# Autodesk Inventor assembly: Base Cover Assembly
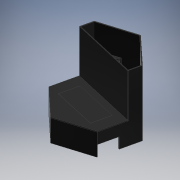
[picture p0: Inventor's stored thumbnail of the model, 180x180]
Saved by Autodesk Inventor 2017 (Build 210142000, 142)
## iProperties
Created: 2018-10-18
Part Number: Base Cover Assembly
Document SubType Name: Assembly
Designer: Dell
Author: Dell
## Documents named in this file (12)
- C:\Users\Dell\Documents\GitHub\tr2\Base\Base Cover Assembly.iam
- C:\Users\Dell\Documents\GitHub\tr2\Base\BA03.ipt
- C:\Users\Dell\Documents\GitHub\tr2\Base\BA04.ipt
- C:\Users\Dell\Documents\GitHub\tr2\Base\BA05.ipt
- C:\Users\Dell\Documents\GitHub\tr2\Base\BA10.ipt
- C:\Users\Dell\Documents\GitHub\tr2\Base\BA14.ipt
- C:\Users\Dell\Documents\GitHub\tr2\Base\BA19.ipt
- C:\Users\Dell\Documents\GitHub\tr2\Base\BA25.ipt
- C:\Users\Dell\Documents\GitHub\tr2\Base\BA26.ipt
- C:\Users\Dell\Documents\GitHub\tr2\Base\BA27.ipt
- C:\Users\Dell\slaterobots.com\Slate Robotics OneDrive - Documents\Autodesk Inventor\tr2-rs1\Base\HDMI Port.ipt
- C:\Users\Dell\slaterobots.com\Slate Robotics OneDrive - Documents\Autodesk Inventor\tr2-rs1\Base\Power Switch\Power Switch.iam
## Components (12 placed, 11 different names)
1. BA04:1 — Mate:7, Mate:8, Flush:1, Flush:4, Mate:12, Flush:8, Mate:22
2. BA05:1 — Mate:5, Mate:6, Flush:3, Mate:13, Mate:20, Flush:9, Mate:21
3. BA03:5 — Flush:2, Flush:3, Mate:18, Mate:21
4. BA10:1 — Mate:3, Mate:4, Mate:6, Mate:8, Flush:7, Mate:14, Mate:15, Mate:16, Mate:17, Mate:20
5. BA14:1 — Flush:1, Flush:2, Mate:18, Mate:22, Mate:23, Mate:24, Mate:25
6. BA19:2 — Flush:4, Mate:12, Mate:13, Flush:8, Flush:9
7. BA25:1 — Mate:1, Mate:4, Mate:7, Mate:17
8. BA25:2 — Mate:1, Mate:3, Mate:5, Mate:16
9. BA26:1 — Flush:7, Mate:14, Mate:15
10. BA27:1 — Mate:23, Mate:24, Mate:25, Mate:26, Mate:27, Angle:1, Mate:28, Mate:29, Flush:10
11. HDMI Port:1 — Mate:28, Mate:29, Flush:10
12. Power Switch:1 [sub-assembly] — Mate:26, Mate:27, Angle:1
## Relationships (33: Mate 24, Flush 8, Angle 1)
- Mate:1: BA25:1 ↔ BA25:2
- Mate:3: BA10:1 ↔ BA25:2
- Mate:4: BA10:1 ↔ BA25:1
- Mate:5: BA05:1 ↔ BA25:2
- Mate:6: BA05:1 ↔ BA10:1
- Mate:7: BA04:1 ↔ BA25:1
- Mate:8: BA04:1 ↔ BA10:1
- Flush:1: BA04:1 ↔ BA14:1
- Flush:2: BA03:5 ↔ BA14:1
- Flush:3: BA05:1 ↔ BA03:5
- Flush:4: BA04:1 ↔ BA19:2
- Mate:12: BA04:1 ↔ BA19:2
- Mate:13: BA05:1 ↔ BA19:2
- Flush:7: BA10:1 ↔ BA26:1
- Mate:14: BA10:1 ↔ BA26:1
- Mate:15 (1 mm): BA10:1 ↔ BA26:1
- Mate:16: BA10:1 ↔ BA25:2
- Mate:17: BA10:1 ↔ BA25:1
- Mate:18: BA03:5 ↔ BA14:1
- Mate:20: BA05:1 ↔ BA10:1
- Flush:8: BA04:1 ↔ BA19:2
- Flush:9: BA05:1 ↔ BA19:2
- Mate:21: BA05:1 ↔ BA03:5
- Mate:22: BA04:1 ↔ BA14:1
- Mate:23: BA14:1 ↔ BA27:1
- Mate:24 (1 mm): BA14:1 ↔ BA27:1
- Mate:25 (1 mm): BA14:1 ↔ BA27:1
- Mate:26: BA27:1 ↔ Power Switch:1
- Mate:27: BA27:1 ↔ Power Switch:1
- Angle:1 (0 deg): BA27:1 ↔ Power Switch:1
- Mate:28 (1 mm): BA27:1 ↔ HDMI Port:1
- Mate:29 (1 mm): BA27:1 ↔ HDMI Port:1
- Flush:10: BA27:1 ↔ HDMI Port:1
